# Autodesk Inventor assembly: Board_V1
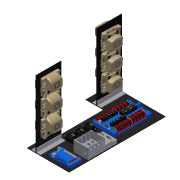
[picture p0: Inventor's stored thumbnail of the model, 180x180]
Saved by Autodesk Inventor 2012 (Build 160160000, 160)
## iProperties
Created: 2012-01-21
Part Number: Board_V1
Document SubType Name: Assembly
Designer: JesseK
Mass: 6803.89 g
Surface Area: 20851.1 cm^2
Volume: 5551.41 cm^3
Density: 1.22561 g/cm^3
Author: JesseK
## Documents named in this file (7)
- Z:\UserData\Documents\Inventor\team1885frc\Robot2012\Electronics Board\Board_V1.iam
- Z:\UserData\Documents\Inventor\team1885frc\Robot2012\Electronics Board\Board_V1.ipt
- Z:\UserData\Documents\Inventor\team1885frc\Electronics\spike relay\Spike_Assem.iam
- Z:\UserData\Documents\Inventor\team1885frc\Electronics\PowerDistributionBoard\elc_Power_Distro_inv.iam
- Z:\UserData\Documents\Inventor\team1885frc\Electronics\DigitalSidecar\elc_Digital_Sidecar_inv.iam
- Z:\UserData\Documents\Inventor\team1885frc\Electronics\cRIO_4Slot\Imported Components\cu_crio-9075_4-slot\cu_crio-9075_4-slot.ipt
- Z:\UserData\Documents\Inventor\team1885frc\Robot2012\Electronics Board\VerticalJagTower.iam
## Components (9 placed, 6 different names)
1. Board_V1:1 — Mate:1, Mate:2, Mate:3, Mate:5, Mate:6, Mate:7, Mate:8, Mate:1, Flush:1, Mate:9, Mate:10, Flush:4, Flush:5
2. Spike_Assem:2 [sub-assembly] — Mate:5
3. Spike_Assem:3 [sub-assembly] — Mate:6
4. Spike_Assem:4 [sub-assembly] — Mate:7
5. elc_Power_Distro_inv:1 [sub-assembly] — Mate:1, Mate:2
6. elc_Digital_Sidecar_inv:1 [sub-assembly] — Mate:3, Flush:1
7. cu_crio-9075_4-slot:1 — Mate:8, Mate:1
8. VerticalJagTower:1 [sub-assembly] — Mate:9, Flush:4
9. VerticalJagTower:2 [sub-assembly] — Mate:10, Flush:5
## Relationships (13: Mate 10, Flush 3)
- Mate:1: Board_V1:1 ↔ elc_Power_Distro_inv:1
- Mate:2 (-38.1 mm): Board_V1:1 ↔ elc_Power_Distro_inv:1
- Mate:3: Board_V1:1 ↔ elc_Digital_Sidecar_inv:1
- Mate:5: Board_V1:1 ↔ Spike_Assem:2
- Mate:6: Board_V1:1 ↔ Spike_Assem:3
- Mate:7: Board_V1:1 ↔ Spike_Assem:4
- Mate:8: Board_V1:1 ↔ cu_crio-9075_4-slot:1
- Mate:1 (-266.7 mm): Board_V1:1 ↔ cu_crio-9075_4-slot:1
- Flush:1 (25.4 mm): Board_V1:1 ↔ elc_Digital_Sidecar_inv:1
- Mate:9: Board_V1:1 ↔ VerticalJagTower:1
- Mate:10: Board_V1:1 ↔ VerticalJagTower:2
- Flush:4: Board_V1:1 ↔ VerticalJagTower:1
- Flush:5: Board_V1:1 ↔ VerticalJagTower:2
